# Autodesk Inventor assembly: R-wing
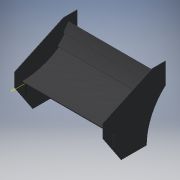
[picture p0: Inventor's stored thumbnail of the model, 180x180]
Saved by Autodesk Inventor 2018.1 (Build 221171000, 171)
## iProperties
Created: 2017-10-27
Part Number: R-wing
Material: 一般
Document SubType Name: Assembly
Designer: kuwano
Mass: 7991.86 g
Surface Area: 36327.8 cm^2
Volume: 5586.99 cm^3
Density: 1.43044 g/cm^3
Author: kuwano
## Documents named in this file (7)
- D:\ku_sk\ドキュメント\Inventor\KS-15_Aero_CAD\type5\R-wing\R-wing.iam
- D:\ku_sk\ドキュメント\Inventor\KS-15_Aero_CAD\type5\R-wing\parts\end_plate.ipt
- D:\ku_sk\ドキュメント\Inventor\KS-15_Aero_CAD\type5\R-wing\parts\element_r_1.ipt
- D:\ku_sk\ドキュメント\Inventor\KS-15_Aero_CAD\type5\R-wing\parts\element_r_2.ipt
- D:\ku_sk\ドキュメント\Inventor\KS-15_Aero_CAD\type5\R-wing\parts\element_clip.ipt
- D:\ku_sk\ドキュメント\Inventor\KS-15_Aero_CAD\type5\R-wing\parts\cover_re.ipt
- D:\ku_sk\ドキュメント\Inventor\KS-15_Aero_CAD\type5\R-wing\parts\end_plate_MIR.ipt
## Components (13 placed, 6 different names)
1. end_plate:2 — メイト:3, メイト:4, メイト:21, メイト:22, メイト:25
2. element_r_1:1 — フラッシュ:1, メイト:3, メイト:9, フラッシュ:7, メイト:10, メイト:11, フラッシュ:8, メイト:12, メイト:13, フラッシュ:9, メイト:14, メイト:15, フラッシュ:10, メイト:16
3. element_r_2:1 — フラッシュ:2, メイト:4, メイト:5, フラッシュ:5, メイト:6, メイト:7, フラッシュ:6, メイト:8, メイト:17, メイト:18, フラッシュ:11, フラッシュ:12, メイト:19, メイト:20
4. cover_re:1 — メイト:25
5. element_clip:1 — メイト:17, フラッシュ:11, メイト:19, メイト:26
6. element_clip:2 — メイト:18, フラッシュ:12, メイト:20
7. element_clip:3 — メイト:9, フラッシュ:7, メイト:10, メイト:22
8. element_clip:4 — メイト:11, フラッシュ:8, メイト:12
9. element_clip:5 — メイト:5, フラッシュ:5, メイト:6, メイト:21
10. element_clip:6 — メイト:7, フラッシュ:6, メイト:8
11. element_clip:7 — メイト:15, フラッシュ:10, メイト:16, メイト:27, メイト:28
12. element_clip:8 — メイト:13, フラッシュ:9, メイト:14
13. end_plate_MIR:1 — メイト:26, メイト:27, メイト:28
## Relationships (34: Mate 24, Flush 10)
- フラッシュ:1 [Flush]: element_r_1:1
- フラッシュ:2 [Flush]: element_r_2:1
- メイト:3 [Mate]: end_plate:2 ↔ element_r_1:1
- メイト:4 [Mate]: end_plate:2 ↔ element_r_2:1
- メイト:5 [Mate]: element_r_2:1 ↔ element_clip:5
- フラッシュ:5 [Flush]: element_r_2:1 ↔ element_clip:5
- メイト:6 [Mate]: element_r_2:1 ↔ element_clip:5
- メイト:7 [Mate]: element_r_2:1 ↔ element_clip:6
- フラッシュ:6 [Flush]: element_r_2:1 ↔ element_clip:6
- メイト:8 [Mate]: element_r_2:1 ↔ element_clip:6
- メイト:9 [Mate]: element_r_1:1 ↔ element_clip:3
- フラッシュ:7 [Flush]: element_r_1:1 ↔ element_clip:3
- メイト:10 [Mate]: element_r_1:1 ↔ element_clip:3
- メイト:11 [Mate]: element_r_1:1 ↔ element_clip:4
- フラッシュ:8 [Flush]: element_r_1:1 ↔ element_clip:4
- メイト:12 [Mate]: element_r_1:1 ↔ element_clip:4
- メイト:13 [Mate]: element_r_1:1 ↔ element_clip:8
- フラッシュ:9 [Flush]: element_r_1:1 ↔ element_clip:8
- メイト:14 [Mate]: element_r_1:1 ↔ element_clip:8
- メイト:15 [Mate]: element_r_1:1 ↔ element_clip:7
- フラッシュ:10 [Flush]: element_r_1:1 ↔ element_clip:7
- メイト:16 [Mate]: element_r_1:1 ↔ element_clip:7
- メイト:17 [Mate]: element_r_2:1 ↔ element_clip:1
- メイト:18 [Mate]: element_r_2:1 ↔ element_clip:2
- フラッシュ:11 [Flush]: element_r_2:1 ↔ element_clip:1
- フラッシュ:12 [Flush]: element_r_2:1 ↔ element_clip:2
- メイト:19 [Mate]: element_r_2:1 ↔ element_clip:1
- メイト:20 [Mate]: element_r_2:1 ↔ element_clip:2
- メイト:21 [Mate]: end_plate:2 ↔ element_clip:5
- メイト:22 [Mate]: end_plate:2 ↔ element_clip:3
- メイト:25 [Mate]: end_plate:2 ↔ cover_re:1
- メイト:26 [Mate]: element_clip:1 ↔ end_plate_MIR:1
- メイト:27 [Mate]: element_clip:7 ↔ end_plate_MIR:1
- メイト:28 [Mate]: element_clip:7 ↔ end_plate_MIR:1
